# Autodesk Inventor assembly: Assembly1
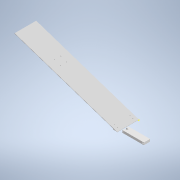
[picture p0: Inventor's stored thumbnail of the model, 180x180]
Saved by Autodesk Inventor 2020 (Build 240168000, 168)
## iProperties
Created: 2021-01-30
Part Number: Assembly1
Document SubType Name: Assembly
Designer: magda
Author: magda
## Documents named in this file (3)
- C:\Users\magda\OneDrive\Documents\Inventor\T3\Ramp Intake\Assembly1.iam
- C:\Users\magda\OneDrive\Documents\Inventor\T3\Ramp Intake\Ramp Base.ipt
- C:\Users\magda\OneDrive\Documents\Inventor\T3\Ramp Intake\Pneumatics Mounted in Undercarriage.iam
## Components (2 placed, 2 different names)
1. Ramp Base:1 — Mate:1, Mate:2
2. Pneumatics Mounted in Undercarriage:1 [sub-assembly] — Mate:1, Mate:2
## Relationships (2: Mate 2)
- Mate:1: Ramp Base:1 ↔ Pneumatics Mounted in Undercarriage:1
- Mate:2: Ramp Base:1 ↔ Pneumatics Mounted in Undercarriage:1
